# Autodesk Inventor assembly: chassis_2
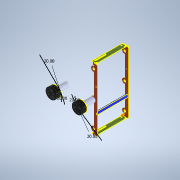
[picture p0: Inventor's stored thumbnail of the model, 180x180]
Saved by Autodesk Inventor 2022 (Build 260153000, 153)
## iProperties
Created: 2023-03-24
Part Number: chassis_2
Document SubType Name: Assembly
Designer: Johnny Jou
Author: Johnny Jou
## Documents named in this file (8)
- C:\Users\Johnny Jou\Documents\GitHub\Areo_Rider_Cabin\car\chassis_2.iam
- C:\Users\Johnny Jou\Documents\GitHub\Areo_Rider_Cabin\car\chassis_1_1.ipt
- C:\Users\Johnny Jou\Documents\GitHub\Areo_Rider_Cabin\car\chassis_1_2.ipt
- C:\Users\Johnny Jou\Documents\GitHub\Areo_Rider_Cabin\car\chassis_1_3.ipt
- C:\Users\Johnny Jou\Documents\GitHub\Areo_Rider_Cabin\car\chassis_1_4.ipt
- C:\Users\Johnny Jou\Documents\GitHub\Areo_Rider_Cabin\motor\25GA370.ipt
- C:\Users\Johnny Jou\Documents\GitHub\Areo_Rider_Cabin\car\Coupling.ipt
- C:\Users\Johnny Jou\Documents\GitHub\Areo_Rider_Cabin\car\wheel.ipt
## Components (12 placed, 7 different names)
1. chassis_1_1:1 — 貼合:1, 貼合:2, 齊平:1, 齊平:4, 貼合:12, 齊平:10
2. chassis_1_2:1 — 貼合:1, 貼合:2, 齊平:1, 貼合:3, 齊平:2, 貼合:4
3. chassis_1_2:2 — 齊平:3, 貼合:5, 貼合:6
4. chassis_1_1:2 — 貼合:3, 齊平:2, 貼合:4, 齊平:3, 貼合:5, 貼合:6, 貼合:7, 貼合:8, 貼合:14, 貼合:15, 貼合:41
5. chassis_1_3:1 — 貼合:7, 貼合:8, 齊平:4
6. chassis_1_4:4 — 貼合:12, 齊平:10
7. 25GA370:3 — 貼合:14, 貼合:15, 貼合:34, 貼合:35
8. Coupling:1 — 貼合:34, 貼合:35
9. wheel:1
10. 25GA370:4 — 貼合:41
11. Coupling:2
12. wheel:2
## Relationships (27: Mate 22, Flush 5)
- 貼合:1 [Mate]: chassis_1_1:1 ↔ chassis_1_2:1
- 貼合:2 [Mate]: chassis_1_1:1 ↔ chassis_1_2:1
- 齊平:1 [Flush]: chassis_1_1:1 ↔ chassis_1_2:1
- 貼合:3 [Mate]: chassis_1_2:1 ↔ chassis_1_1:2
- 齊平:2 [Flush]: chassis_1_2:1 ↔ chassis_1_1:2
- 貼合:4 [Mate]: chassis_1_2:1 ↔ chassis_1_1:2
- 齊平:3 [Flush]: chassis_1_2:2 ↔ chassis_1_1:2
- 貼合:5 [Mate]: chassis_1_2:2 ↔ chassis_1_1:2
- 貼合:6 [Mate]: chassis_1_2:2 ↔ chassis_1_1:2
- 貼合:7 [Mate]: chassis_1_1:2 ↔ chassis_1_3:1
- 貼合:8 [Mate]: chassis_1_1:2 ↔ chassis_1_3:1
- 齊平:4 [Flush]: chassis_1_1:1 ↔ chassis_1_3:1
- 貼合:12 [Mate]: chassis_1_1:1 ↔ chassis_1_4:4
- 齊平:10 [Flush]: chassis_1_1:1 ↔ chassis_1_4:4
- 貼合:14 [Mate]: chassis_1_1:2 ↔ 25GA370:3
- 貼合:15 [Mate]: chassis_1_1:2 ↔ 25GA370:3
- [Mate]: Coupling:1 ↔ wheel:1
- [Mate]: Coupling:1 ↔ wheel:1
- [Mate]: Coupling:1 ↔ wheel:1
- 貼合:34 [Mate]: 25GA370:3 ↔ Coupling:1
- 貼合:35 [Mate]: 25GA370:3 ↔ Coupling:1
- [Mate]: Coupling:2 ↔ wheel:2
- [Mate]: Coupling:2 ↔ wheel:2
- [Mate]: Coupling:2 ↔ wheel:2
- [Mate]: 25GA370:4 ↔ Coupling:2
- [Mate]: 25GA370:4 ↔ Coupling:2
- 貼合:41 [Mate]: chassis_1_1:2 ↔ 25GA370:4
## Named parameters: d32_d21 = 0 mm, d33_d22 = 0 mm, d34_d23 = 0 mm, d60_d32_d21 = 0 mm, d61_d33_d22 = 0 mm, d62_d34_d23 = 0 mm, d63_d58 = 0 mm, d64_d59 = 0 mm
